# Autodesk Inventor assembly: Assieme1
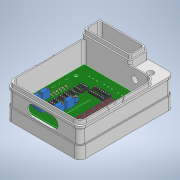
[picture p0: Inventor's stored thumbnail of the model, 180x180]
Saved by Autodesk Inventor 2021 (Build 250183000, 183)
## iProperties
Created: 2021-10-08
Part Number: Assieme1
Document SubType Name: Assembly
Designer: Matteo
Author: Matteo
## Documents named in this file (3)
- C:\Users\Matteo\Desktop\UNITN\Tesi\Custodia\last version\Assieme1.iam
- C:\Users\Matteo\Desktop\UNITN\Tesi\Custodia\last version\Parte1.ipt
- C:\Users\Matteo\Desktop\UNITN\Tesi\Custodia\last version\PCB_Definitivo.iam
## Components (2 placed, 2 different names)
1. Parte1:1 — Coincidente:1, Coincidente:2, Coincidente:3
2. PCB_Definitivo:1 [sub-assembly] — Coincidente:1, Coincidente:2, Coincidente:3
## Relationships (3: Mate 3)
- Coincidente:1 [Mate] (13 mm): Parte1:1 ↔ PCB_Definitivo:1
- Coincidente:2 [Mate] (2.542 mm): Parte1:1 ↔ PCB_Definitivo:1
- Coincidente:3 [Mate] (3.09 mm): Parte1:1 ↔ PCB_Definitivo:1
